# Autodesk Inventor assembly: 06-01-2023 assieme Verifica
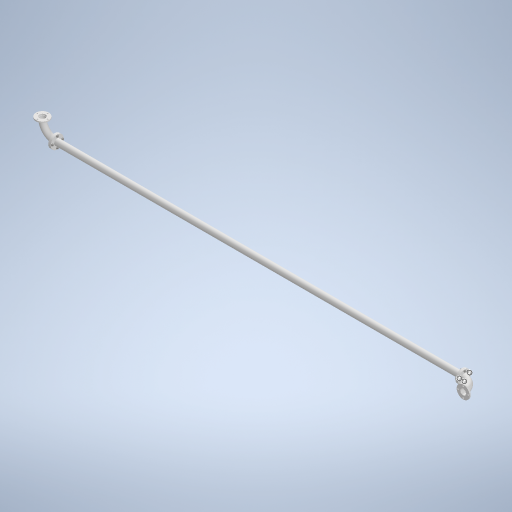
[picture p0: Inventor's stored thumbnail of the model, 512x512]
Saved by Autodesk Inventor 2023 (Build 270158000, 158)
## iProperties
Created: 2023-06-01
Part Number: 06-01-2023 assieme Verifica
Document SubType Name: Assembly
Designer: Admin
Author: Admin
## Documents named in this file (7)
- C:\Users\Admin\Desktop\3DDDD\06-01-2023 assieme Verifica.iam
- C:\Users\Admin\Desktop\3DDDD\06-01-2023 flangia DN80.ipt
- C:\Users\Admin\Desktop\3DDDD\06-01-2023 Verga 88,9.ipt
- C:\Users\Admin\Desktop\3DDDD\06-01-2023 curva 90° R200.ipt
- C:\Users\Admin\Documents\Inventor\Content Center Files\R2023\it-IT\BS EN ISO 4015\BS EN ISO 4015 - M16x55.ipt
- C:\Users\Admin\Documents\Inventor\Content Center Files\R2023\it-IT\IS 2016  A\IS 2016 - A20.ipt
- C:\Users\Admin\Documents\Inventor\Content Center Files\R2023\it-IT\CSN EN 24035\ISO 4035 - M16CSN EN.ipt
## Components (33 placed, 6 different names)
1. 06-01-2023 flangia DN80:1 — Allineato:1, Coincidente:1, Coincidente:2, Coincidente:3, Coincidente:4, Coincidente:5, Coincidente:6, Allineato:5, Coincidente:29, Coincidente:30, Coincidente:31, Inserimento:6, Inserimento:7, Inserimento:8, Inserimento:9, Coincidente:60, Coincidente:61, Coincidente:62, Coincidente:63, Coincidente:64, Coincidente:65, Coincidente:66, Coincidente:67
2. 06-01-2023 Verga 88,9:1 — Allineato:1, Coincidente:1, Coincidente:2, Coincidente:7, Allineato:3, Coincidente:11, Coincidente:17
3. 06-01-2023 flangia DN80:2 — Coincidente:3, Coincidente:4, Coincidente:5, Coincidente:8, Inserimento:2, Inserimento:3, Inserimento:4, Inserimento:5
4. 06-01-2023 curva 90° R200:1 — Coincidente:6, Coincidente:7, Coincidente:8, Allineato:2, Coincidente:9, Coincidente:10
5. 06-01-2023 flangia DN80:3 — Allineato:2, Coincidente:9, Coincidente:10
6. 06-01-2023 flangia DN80:4 — Allineato:3, Coincidente:11, Coincidente:14, Coincidente:15, Coincidente:16, Coincidente:17, Coincidente:32, Coincidente:33, Coincidente:34, Coincidente:35, Inserimento:10, Inserimento:11, Inserimento:12, Inserimento:13, Coincidente:37, Coincidente:52, Coincidente:53, Coincidente:54, Coincidente:55, Coincidente:56, Coincidente:57, Coincidente:58, Coincidente:59
7. 06-01-2023 flangia DN80:5 — Allineato:4, Coincidente:13, Coincidente:14, Coincidente:15, Coincidente:16, Coincidente:18, Coincidente:21, Coincidente:22, Coincidente:23, Coincidente:24, Coincidente:25, Coincidente:26, Coincidente:27, Coincidente:28
8. 06-01-2023 flangia DN80:6 — Coincidente:20, Inserimento:1
9. 06-01-2023 curva 90° R200:2 — Allineato:4, Coincidente:13, Coincidente:18, Coincidente:20, Inserimento:1
10. BS EN ISO 4015 M16x55:1 — Inserimento:2, Allineato:5, Coincidente:48
11. BS EN ISO 4015 M16x55:2 — Inserimento:3, Coincidente:29, Coincidente:44
12. BS EN ISO 4015 M16x55:3 — Inserimento:4, Coincidente:30, Coincidente:46
13. BS EN ISO 4015 M16x55:4 — Inserimento:5, Coincidente:31, Coincidente:50
14. BS EN ISO 4015 M16x55:5 — Coincidente:21, Coincidente:22, Coincidente:32, Coincidente:38
15. BS EN ISO 4015 M16x55:6 — Coincidente:23, Coincidente:24, Coincidente:34, Coincidente:36
16. BS EN ISO 4015 M16x55:7 — Coincidente:25, Coincidente:26, Coincidente:33, Coincidente:42
17. BS EN ISO 4015 M16x55:8 — Coincidente:27, Coincidente:28, Coincidente:35, Coincidente:40
18. IS 2016 A A20:1 — Inserimento:6, Coincidente:51, Coincidente:62
19. IS 2016 A A20:2 — Inserimento:7, Coincidente:45, Coincidente:60
20. IS 2016 A A20:3 — Inserimento:8, Coincidente:49, Coincidente:61
21. IS 2016 A A20:4 — Inserimento:9, Coincidente:47, Coincidente:63
22. IS 2016 A A20:5 — Inserimento:10, Coincidente:41, Coincidente:52
23. IS 2016 A A20:6 — Inserimento:11, Coincidente:39, Coincidente:54
24. IS 2016 A A20:7 — Inserimento:12, Coincidente:53
25. IS 2016 A A20:8 — Inserimento:13, Coincidente:43, Coincidente:55
26. CSN EN 24035 M16:1 — Coincidente:36, Coincidente:37, Coincidente:56
27. CSN EN 24035 M16:2 — Coincidente:38, Coincidente:39, Coincidente:58
28. CSN EN 24035 M16:3 — Coincidente:40, Coincidente:41, Coincidente:57
29. CSN EN 24035 M16:4 — Coincidente:42, Coincidente:43, Coincidente:59
30. CSN EN 24035 M16:5 — Coincidente:44, Coincidente:45, Coincidente:64
31. CSN EN 24035 M16:6 — Coincidente:46, Coincidente:47, Coincidente:65
32. CSN EN 24035 M16:7 — Coincidente:48, Coincidente:49, Coincidente:67
33. CSN EN 24035 M16:8 — Coincidente:50, Coincidente:51, Coincidente:66
## Relationships (83: Mate 65, Insert 13, Flush 5)
- Allineato:1 [Flush]: 06-01-2023 flangia DN80:1 ↔ 06-01-2023 Verga 88,9:1
- Coincidente:1 [Mate]: 06-01-2023 flangia DN80:1 ↔ 06-01-2023 Verga 88,9:1
- Coincidente:2 [Mate]: 06-01-2023 flangia DN80:1 ↔ 06-01-2023 Verga 88,9:1
- Coincidente:3 [Mate]: 06-01-2023 flangia DN80:1 ↔ 06-01-2023 flangia DN80:2
- Coincidente:4 [Mate]: 06-01-2023 flangia DN80:1 ↔ 06-01-2023 flangia DN80:2
- Coincidente:5 [Mate]: 06-01-2023 flangia DN80:1 ↔ 06-01-2023 flangia DN80:2
- Coincidente:6 [Mate]: 06-01-2023 flangia DN80:1 ↔ 06-01-2023 curva 90° R200:1
- Coincidente:7 [Mate]: 06-01-2023 Verga 88,9:1 ↔ 06-01-2023 curva 90° R200:1
- Coincidente:8 [Mate]: 06-01-2023 flangia DN80:2 ↔ 06-01-2023 curva 90° R200:1
- Allineato:2 [Flush]: 06-01-2023 curva 90° R200:1 ↔ 06-01-2023 flangia DN80:3
- Coincidente:9 [Mate]: 06-01-2023 curva 90° R200:1 ↔ 06-01-2023 flangia DN80:3
- Coincidente:10 [Mate]: 06-01-2023 curva 90° R200:1 ↔ 06-01-2023 flangia DN80:3
- Allineato:3 [Flush]: 06-01-2023 Verga 88,9:1 ↔ 06-01-2023 flangia DN80:4
- Coincidente:11 [Mate]: 06-01-2023 Verga 88,9:1 ↔ 06-01-2023 flangia DN80:4
- Allineato:4 [Flush]: 06-01-2023 flangia DN80:5 ↔ 06-01-2023 curva 90° R200:2
- Coincidente:13 [Mate]: 06-01-2023 flangia DN80:5 ↔ 06-01-2023 curva 90° R200:2
- Coincidente:14 [Mate]: 06-01-2023 flangia DN80:4 ↔ 06-01-2023 flangia DN80:5
- Coincidente:15 [Mate]: 06-01-2023 flangia DN80:4 ↔ 06-01-2023 flangia DN80:5
- Coincidente:16 [Mate]: 06-01-2023 flangia DN80:4 ↔ 06-01-2023 flangia DN80:5
- Coincidente:17 [Mate]: 06-01-2023 Verga 88,9:1 ↔ 06-01-2023 flangia DN80:4
- Coincidente:18 [Mate]: 06-01-2023 flangia DN80:5 ↔ 06-01-2023 curva 90° R200:2
- Coincidente:20 [Mate]: 06-01-2023 flangia DN80:6 ↔ 06-01-2023 curva 90° R200:2
- Inserimento:1: 06-01-2023 flangia DN80:6 ↔ 06-01-2023 curva 90° R200:2
- Inserimento:2: 06-01-2023 flangia DN80:2 ↔ BS EN ISO 4015 M16x55:1
- Inserimento:3: 06-01-2023 flangia DN80:2 ↔ BS EN ISO 4015 M16x55:2
- Inserimento:4: 06-01-2023 flangia DN80:2 ↔ BS EN ISO 4015 M16x55:3
- Inserimento:5: 06-01-2023 flangia DN80:2 ↔ BS EN ISO 4015 M16x55:4
- Coincidente:21 [Mate]: 06-01-2023 flangia DN80:5 ↔ BS EN ISO 4015 M16x55:5
- Coincidente:22 [Mate]: 06-01-2023 flangia DN80:5 ↔ BS EN ISO 4015 M16x55:5
- Coincidente:23 [Mate]: 06-01-2023 flangia DN80:5 ↔ BS EN ISO 4015 M16x55:6
- Coincidente:24 [Mate]: 06-01-2023 flangia DN80:5 ↔ BS EN ISO 4015 M16x55:6
- Coincidente:25 [Mate]: 06-01-2023 flangia DN80:5 ↔ BS EN ISO 4015 M16x55:7
- Coincidente:26 [Mate]: 06-01-2023 flangia DN80:5 ↔ BS EN ISO 4015 M16x55:7
- Coincidente:27 [Mate]: 06-01-2023 flangia DN80:5 ↔ BS EN ISO 4015 M16x55:8
- Coincidente:28 [Mate]: 06-01-2023 flangia DN80:5 ↔ BS EN ISO 4015 M16x55:8
- Allineato:5 [Flush]: 06-01-2023 flangia DN80:1 ↔ BS EN ISO 4015 M16x55:1
- Coincidente:29 [Mate]: 06-01-2023 flangia DN80:1 ↔ BS EN ISO 4015 M16x55:2
- Coincidente:30 [Mate]: 06-01-2023 flangia DN80:1 ↔ BS EN ISO 4015 M16x55:3
- Coincidente:31 [Mate]: 06-01-2023 flangia DN80:1 ↔ BS EN ISO 4015 M16x55:4
- Coincidente:32 [Mate]: 06-01-2023 flangia DN80:4 ↔ BS EN ISO 4015 M16x55:5
- Coincidente:33 [Mate]: 06-01-2023 flangia DN80:4 ↔ BS EN ISO 4015 M16x55:7
- Coincidente:34 [Mate]: 06-01-2023 flangia DN80:4 ↔ BS EN ISO 4015 M16x55:6
- Coincidente:35 [Mate]: 06-01-2023 flangia DN80:4 ↔ BS EN ISO 4015 M16x55:8
- Inserimento:6: 06-01-2023 flangia DN80:1 ↔ IS 2016 A A20:1
- Inserimento:7: 06-01-2023 flangia DN80:1 ↔ IS 2016 A A20:2
- Inserimento:8: 06-01-2023 flangia DN80:1 ↔ IS 2016 A A20:3
- Inserimento:9: 06-01-2023 flangia DN80:1 ↔ IS 2016 A A20:4
- Inserimento:10: 06-01-2023 flangia DN80:4 ↔ IS 2016 A A20:5
- Inserimento:11: 06-01-2023 flangia DN80:4 ↔ IS 2016 A A20:6
- Inserimento:12: 06-01-2023 flangia DN80:4 ↔ IS 2016 A A20:7
- Inserimento:13: 06-01-2023 flangia DN80:4 ↔ IS 2016 A A20:8
- Coincidente:36 [Mate]: BS EN ISO 4015 M16x55:6 ↔ CSN EN 24035 M16:1
- Coincidente:37 [Mate]: 06-01-2023 flangia DN80:4 ↔ CSN EN 24035 M16:1
- Coincidente:38 [Mate]: BS EN ISO 4015 M16x55:5 ↔ CSN EN 24035 M16:2
- Coincidente:39 [Mate]: IS 2016 A A20:6 ↔ CSN EN 24035 M16:2
- Coincidente:40 [Mate]: BS EN ISO 4015 M16x55:8 ↔ CSN EN 24035 M16:3
- Coincidente:41 [Mate]: IS 2016 A A20:5 ↔ CSN EN 24035 M16:3
- Coincidente:42 [Mate]: BS EN ISO 4015 M16x55:7 ↔ CSN EN 24035 M16:4
- Coincidente:43 [Mate]: IS 2016 A A20:8 ↔ CSN EN 24035 M16:4
- Coincidente:44 [Mate]: BS EN ISO 4015 M16x55:2 ↔ CSN EN 24035 M16:5
- Coincidente:45 [Mate]: IS 2016 A A20:2 ↔ CSN EN 24035 M16:5
- Coincidente:46 [Mate]: BS EN ISO 4015 M16x55:3 ↔ CSN EN 24035 M16:6
- Coincidente:47 [Mate]: IS 2016 A A20:4 ↔ CSN EN 24035 M16:6
- Coincidente:48 [Mate]: BS EN ISO 4015 M16x55:1 ↔ CSN EN 24035 M16:7
- Coincidente:49 [Mate]: IS 2016 A A20:3 ↔ CSN EN 24035 M16:7
- Coincidente:50 [Mate]: BS EN ISO 4015 M16x55:4 ↔ CSN EN 24035 M16:8
- Coincidente:51 [Mate]: IS 2016 A A20:1 ↔ CSN EN 24035 M16:8
- Coincidente:52 [Mate]: 06-01-2023 flangia DN80:4 ↔ IS 2016 A A20:5
- Coincidente:53 [Mate]: 06-01-2023 flangia DN80:4 ↔ IS 2016 A A20:7
- Coincidente:54 [Mate]: 06-01-2023 flangia DN80:4 ↔ IS 2016 A A20:6
- Coincidente:55 [Mate]: 06-01-2023 flangia DN80:4 ↔ IS 2016 A A20:8
- Coincidente:56 [Mate]: 06-01-2023 flangia DN80:4 ↔ CSN EN 24035 M16:1
- Coincidente:57 [Mate]: 06-01-2023 flangia DN80:4 ↔ CSN EN 24035 M16:3
- Coincidente:58 [Mate]: 06-01-2023 flangia DN80:4 ↔ CSN EN 24035 M16:2
- Coincidente:59 [Mate]: 06-01-2023 flangia DN80:4 ↔ CSN EN 24035 M16:4
- Coincidente:60 [Mate]: 06-01-2023 flangia DN80:1 ↔ IS 2016 A A20:2
- Coincidente:61 [Mate]: 06-01-2023 flangia DN80:1 ↔ IS 2016 A A20:3
- Coincidente:62 [Mate]: 06-01-2023 flangia DN80:1 ↔ IS 2016 A A20:1
- Coincidente:63 [Mate]: 06-01-2023 flangia DN80:1 ↔ IS 2016 A A20:4
- Coincidente:64 [Mate]: 06-01-2023 flangia DN80:1 ↔ CSN EN 24035 M16:5
- Coincidente:65 [Mate]: 06-01-2023 flangia DN80:1 ↔ CSN EN 24035 M16:6
- Coincidente:66 [Mate]: 06-01-2023 flangia DN80:1 ↔ CSN EN 24035 M16:8
- Coincidente:67 [Mate]: 06-01-2023 flangia DN80:1 ↔ CSN EN 24035 M16:7
